# Autodesk Inventor assembly: TC-10012
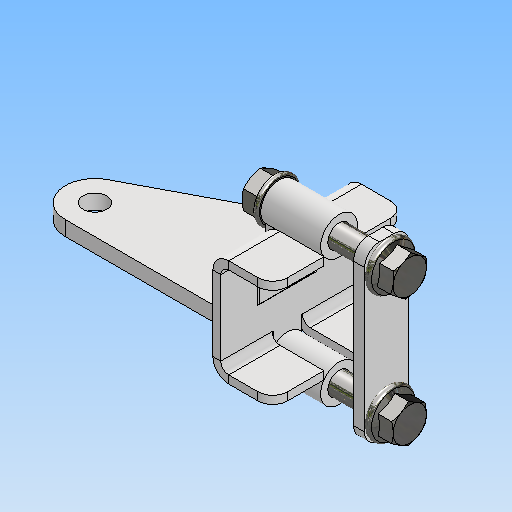
[picture p0: Inventor's stored thumbnail of the model, 512x512]
Saved by Autodesk Inventor 2025.4 (Build 294407000, 407)
## iProperties
Created: 2025-11-28
Part Number: TC-10012
Document SubType Name: Assembly
Designer: josh
Description: 1-1/2" Sq Tube Bolt-on Clamp
Author: josh
## Documents named in this file (7)
- R:\A1- Neuweg Design Data\OM Robotics\CLEANING ROBOT TOWER PROJECT\TC-10012.iam
- R:\A1- Neuweg Design Data\OM Robotics\CLEANING ROBOT TOWER PROJECT\TC-1002.ipt
- R:\A1- Neuweg Design Data\OM Robotics\CLEANING ROBOT TOWER PROJECT\TC-1003.ipt
- R:\A1- Neuweg Design Data\OM Robotics\CLEANING ROBOT TOWER PROJECT\TC-1005.ipt
- R:\A1- Neuweg Design Data\OM Robotics\CLEANING ROBOT TOWER PROJECT\TC-1006.ipt
- R:\A1- Neuweg Design Data\OM Robotics\CLEANING ROBOT TOWER PROJECT\92979A186.ipt
- R:\A1- Neuweg Design Data\OM Robotics\CLEANING ROBOT TOWER PROJECT\94842A103.ipt
## Components (9 placed, 6 different names)
1. TC-1005:1 — Flush:10, Flush:11, Flush:12, Insert:1, Insert:2
2. TC-1003:1 — Flush:7, Flush:8, Flush:9, Mate:4
3. TC-1002:1 — Flush:4, Flush:5, Flush:6
4. TC-1003:2 — Flush:13, Mate:1, Mate:2, Insert:3
5. 92979A186:3 — Insert:1, Mate:3
6. 92979A186:4 — Insert:2
7. 94842A103:3 — Mate:3, Mate:4
8. 94842A103:4 — Insert:3
9. TC-1006:1
## Relationships (17: Flush 10, Mate 4, Insert 3)
- Flush:4: TC-1002:1
- Flush:5: TC-1002:1
- Flush:6: TC-1002:1
- Flush:7: TC-1003:1
- Flush:8: TC-1003:1
- Flush:9: TC-1003:1
- Flush:10: TC-1005:1
- Flush:11: TC-1005:1
- Flush:12: TC-1005:1
- Flush:13: TC-1003:2
- Mate:1: TC-1003:2
- Mate:2: TC-1003:2
- Insert:1: TC-1005:1 ↔ 92979A186:3
- Insert:2: TC-1005:1 ↔ 92979A186:4
- Mate:3: 92979A186:3 ↔ 94842A103:3
- Mate:4: TC-1003:1 ↔ 94842A103:3
- Insert:3: TC-1003:2 ↔ 94842A103:4
